# Autodesk Inventor assembly: Leg
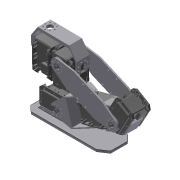
[picture p0: Inventor's stored thumbnail of the model, 180x180]
Saved by Autodesk Inventor 2011 (Build 150239000, 239)
## iProperties
Created: 2010-12-02
Part Number: Leg
Document SubType Name: Assembly
Designer: Milton
Author: Milton
## Documents named in this file (8)
- C:\Users\Milton\Documents\Futbots\IC - Humanóide\Desenhos\Leg.iam
- C:\Users\Milton\Documents\Futbots\IC - Humanóide\Imagens\Imported Components\RX-28 Horn\RX-28 Horn.ipt
- C:\Users\Milton\Documents\Futbots\IC - Humanóide\Desenhos\Thigh.ipt
- C:\Users\Milton\Documents\Futbots\IC - Humanóide\Desenhos\Knee - Front.ipt
- C:\Users\Milton\Documents\Futbots\IC - Humanóide\Desenhos\Knee - Back.ipt
- C:\Users\Milton\Documents\Futbots\IC - Humanóide\Desenhos\Hips.ipt
- C:\Users\Milton\Documents\Futbots\IC - Humanóide\Desenhos\Ankle.ipt
- C:\Users\Milton\Documents\Futbots\IC - Humanóide\Desenhos\Left foot.ipt
## Components (12 placed, 7 different names)
1. RX-28 Horn:1 — Flush:1, Mate:24, Flush:2, Mate:25, Mate:26
2. RX-28 Horn:2 — Mate:19, Mate:20, Mate:23, Flush:1, Mate:24, Flush:2
3. Thigh:1 — Mate:21, Mate:22, Mate:23
4. Knee - Front:1 — Mate:11, Mate:12, Mate:13, Mate:14, Mate:16
5. Knee - Back:1 — Mate:8, Mate:9, Mate:10, Mate:15
6. Thigh:2 — Mate:17, Mate:18, Mate:19, Mate:20
7. Hips:1 — Mate:25, Mate:26
8. RX-28 Horn:3 — Mate:14, Mate:15, Mate:16, Mate:17, Mate:18, Mate:21, Mate:22
9. RX-28 Horn:4 — Mate:1, Mate:2, Mate:3, Mate:4, Mate:5
10. Ankle:1 — Mate:4, Mate:5, Mate:6, Mate:7
11. Left foot:1 — Mate:1, Mate:2, Mate:3
12. RX-28 Horn:5 — Mate:6, Mate:7, Mate:8, Mate:9, Mate:10, Mate:11, Mate:12, Mate:13
## Relationships (28: Mate 26, Flush 2)
- Mate:1: RX-28 Horn:4 ↔ Left foot:1
- Mate:2: RX-28 Horn:4 ↔ Left foot:1
- Mate:3: RX-28 Horn:4 ↔ Left foot:1
- Mate:4: RX-28 Horn:4 ↔ Ankle:1
- Mate:5: RX-28 Horn:4 ↔ Ankle:1
- Mate:6: Ankle:1 ↔ RX-28 Horn:5
- Mate:7: Ankle:1 ↔ RX-28 Horn:5
- Mate:8: Knee - Back:1 ↔ RX-28 Horn:5
- Mate:9: Knee - Back:1 ↔ RX-28 Horn:5
- Mate:10: Knee - Back:1 ↔ RX-28 Horn:5
- Mate:11: Knee - Front:1 ↔ RX-28 Horn:5
- Mate:12: Knee - Front:1 ↔ RX-28 Horn:5
- Mate:13: Knee - Front:1 ↔ RX-28 Horn:5
- Mate:14: Knee - Front:1 ↔ RX-28 Horn:3
- Mate:15: Knee - Back:1 ↔ RX-28 Horn:3
- Mate:16: Knee - Front:1 ↔ RX-28 Horn:3
- Mate:17: Thigh:2 ↔ RX-28 Horn:3
- Mate:18: Thigh:2 ↔ RX-28 Horn:3
- Mate:19: RX-28 Horn:2 ↔ Thigh:2
- Mate:20: RX-28 Horn:2 ↔ Thigh:2
- Mate:21: Thigh:1 ↔ RX-28 Horn:3
- Mate:22: Thigh:1 ↔ RX-28 Horn:3
- Mate:23: RX-28 Horn:2 ↔ Thigh:1
- Flush:1: RX-28 Horn:1 ↔ RX-28 Horn:2
- Mate:24: RX-28 Horn:1 ↔ RX-28 Horn:2
- Flush:2: RX-28 Horn:1 ↔ RX-28 Horn:2
- Mate:25: RX-28 Horn:1 ↔ Hips:1
- Mate:26: RX-28 Horn:1 ↔ Hips:1
